# Autodesk Inventor assembly: PS20026
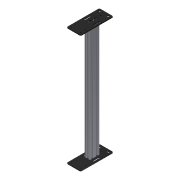
[picture p0: Inventor's stored thumbnail of the model, 180x180]
Saved by Autodesk Inventor 2014 (Build 180170000, 170)
## iProperties
Created: 2013-09-18
Part Number: PS20026
Document SubType Name: Assembly
Designer: Edward
Description: Y-Axis Rail Assembly
Author: Edward
Title: Y-Axis Rail Assembly
Subject: Shapeoko 2
## Documents named in this file (6)
- C:\Users\Edward\Documents\GitHub\Shapeoko_2\Autodesk_Inventor_Project\PS20026.iam
- C:\Users\Edward\Documents\GitHub\Shapeoko_2\Autodesk_Inventor_Project\26028-01.ipt
- C:\Users\Edward\Documents\GitHub\Shapeoko_2\Autodesk_Inventor_Project\25286-02.ipt
- C:\Users\Edward\Documents\GitHub\Shapeoko_2\Autodesk_Inventor_Project\25287-02.ipt
- C:\Users\Edward\Documents\GitHub\Shapeoko_2\Autodesk_Inventor_Project\PS20020.iam
- C:\Users\Edward\Documents\GitHub\Shapeoko_2\Autodesk_Inventor_Project\PS20008.ipt
## Components (13 placed, 5 different names)
1. PS20008:1
2. 26028-01:1
3. 26028-01:2
4. 25286-02:1
5. 25287-02:1
6. 25286-02:2
7. 25287-02:2
8. 25286-02:3
9. 25287-02:3
10. 25286-02:4
11. 25287-02:4
12. PS20020:1 [sub-assembly]
13. PS20020:2 [sub-assembly]
## Relationships (18: Insert 10, Mate 4, Angle 2, Flush 2)
- [Insert]: PS20008:1 ↔ 26028-01:2
- [Insert]: PS20008:1 ↔ 26028-01:1
- [Angle] (0 deg): 26028-01:1 ↔ 26028-01:2
- [Angle] (0 deg): PS20008:1 ↔ 26028-01:2
- [Insert]: 25286-02:1 ↔ 25287-02:1
- [Insert]: 25286-02:2 ↔ 25287-02:2
- [Insert] (3.4163 mm): PS20008:1 ↔ 25287-02:2
- [Insert] (3.4163 mm): PS20008:1 ↔ 25287-02:1
- [Insert]: 25286-02:3 ↔ 25287-02:3
- [Insert]: 25286-02:4 ↔ 25287-02:4
- [Insert]: 26028-01:1 ↔ 25287-02:4
- [Insert] (3.4163 mm): PS20008:1 ↔ 25287-02:3
- [Mate]: PS20008:1 ↔ PS20020:2
- [Mate]: 26028-01:1 ↔ PS20020:2
- [Flush] (3 mm): PS20008:1 ↔ PS20020:2
- [Mate]: PS20008:1 ↔ PS20020:1
- [Flush] (3 mm): PS20008:1 ↔ PS20020:1
- [Mate]: 26028-01:2 ↔ PS20020:1
## Named parameters: d52_d51 = 0 mm, d79_d51 = 0 mm, d80_d51 = 0 mm, d16_d18 = 0 mm
